# Autodesk Inventor assembly: CarrierAxisY
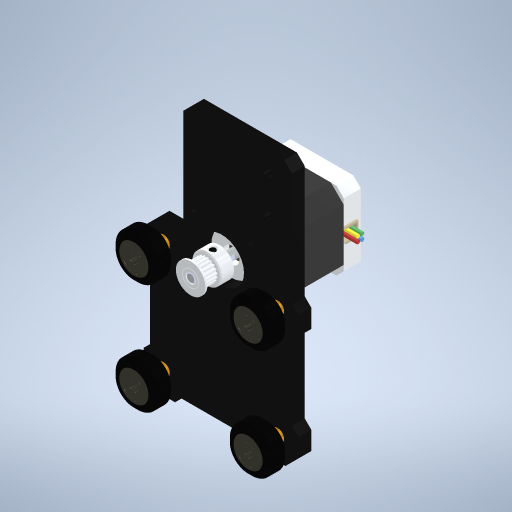
[picture p0: Inventor's stored thumbnail of the model, 512x512]
Saved by Autodesk Inventor 2024.2 (Build 282272000, 272)
## iProperties
Created: 2026-04-14
Part Number: CarrierAxisY
Document SubType Name: Assembly
Designer: Admin
Author: Admin
## Documents named in this file (6)
- C:\Users\Admin\Documents\GitHub\ManipuladorCartesiano\DiseñoMecánico\Assemblies\CarrierAxisY.iam
- C:\Users\Admin\Documents\GitHub\ManipuladorCartesiano\DiseñoMecánico\AcrylicPieces\AxisY-Carrier.ipt
- C:\Users\Admin\Documents\GitHub\ManipuladorCartesiano\DiseñoMecánico\Motors\NEMA17 [48mm]\NEMA17 [48mm].ipt
- C:\Users\Admin\Documents\GitHub\ManipuladorCartesiano\DiseñoMecánico\AuxiliarPieces\Pulley\GT2_20T\GT2_20T.ipt
- C:\Users\Admin\Documents\GitHub\ManipuladorCartesiano\DiseñoMecánico\AuxiliarPieces\M5x6-Insert\M5x6-Insert.ipt
- C:\Users\Admin\Documents\GitHub\ManipuladorCartesiano\DiseñoMecánico\AuxiliarPieces\Bearings\625ZZ\NylonPulleyBearing.iam
## Components (11 placed, 5 different names)
1. AxisY-Carrier:1 — Mate:1, Mate:2, Mate:3, Mate:12, Mate:13, Mate:14, Mate:15, Mate:16, Mate:17, Mate:18, Mate:19
2. NEMA17 [48mm]:1 — Mate:1, Mate:2, Mate:3, Mate:20, Flush:1
3. GT2_20T:1 — Mate:20, Flush:1
4. M5x6-Insert:2 — Mate:4, Mate:5, Mate:15
5. NylonPulleyBearing:1 [sub-assembly] — Mate:4, Mate:5, Mate:14
6. M5x6-Insert:3 — Mate:12
7. NylonPulleyBearing:2 [sub-assembly] — Mate:13
8. M5x6-Insert:4 — Mate:17
9. NylonPulleyBearing:3 [sub-assembly] — Mate:19
10. M5x6-Insert:5 — Mate:16
11. NylonPulleyBearing:4 [sub-assembly] — Mate:18
## Relationships (21: Mate 20, Flush 1)
- Mate:1: AxisY-Carrier:1 ↔ NEMA17 [48mm]:1
- Mate:2: AxisY-Carrier:1 ↔ NEMA17 [48mm]:1
- Mate:3: AxisY-Carrier:1 ↔ NEMA17 [48mm]:1
- Mate:4: M5x6-Insert:2 ↔ NylonPulleyBearing:1
- Mate:5: M5x6-Insert:2 ↔ NylonPulleyBearing:1
- [Mate]: M5x6-Insert:3 ↔ NylonPulleyBearing:2
- [Mate]: M5x6-Insert:3 ↔ NylonPulleyBearing:2
- [Mate]: M5x6-Insert:4 ↔ NylonPulleyBearing:3
- [Mate]: M5x6-Insert:4 ↔ NylonPulleyBearing:3
- [Mate]: M5x6-Insert:5 ↔ NylonPulleyBearing:4
- [Mate]: M5x6-Insert:5 ↔ NylonPulleyBearing:4
- Mate:12: AxisY-Carrier:1 ↔ M5x6-Insert:3
- Mate:13: AxisY-Carrier:1 ↔ NylonPulleyBearing:2
- Mate:14: AxisY-Carrier:1 ↔ NylonPulleyBearing:1
- Mate:15: AxisY-Carrier:1 ↔ M5x6-Insert:2
- Mate:16: AxisY-Carrier:1 ↔ M5x6-Insert:5
- Mate:17: AxisY-Carrier:1 ↔ M5x6-Insert:4
- Mate:18: AxisY-Carrier:1 ↔ NylonPulleyBearing:4
- Mate:19: AxisY-Carrier:1 ↔ NylonPulleyBearing:3
- Mate:20: NEMA17 [48mm]:1 ↔ GT2_20T:1
- Flush:1: NEMA17 [48mm]:1 ↔ GT2_20T:1
## Named parameters: d5_d3 = 0 mm, d6_d4 = 0 mm, d7_d3 = 0 mm, d8_d4 = 0 mm, d9_d3 = 0 mm, d10_d4 = 0 mm
